# Autodesk Inventor assembly: BG102_trajan20_22
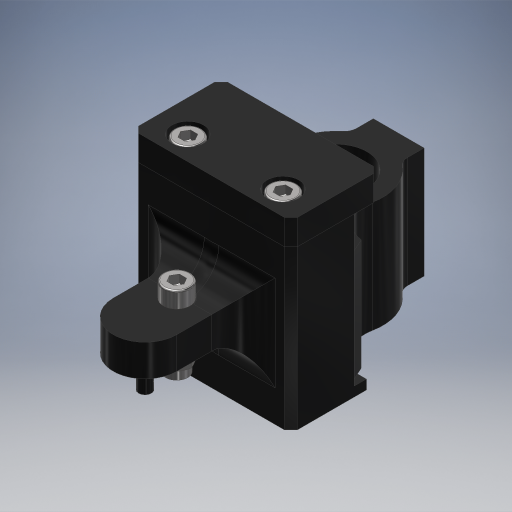
[picture p0: Inventor's stored thumbnail of the model, 512x512]
Saved by Autodesk Inventor 2023 (Build 270158000, 158)
## iProperties
Company: HTBLA Kaindorf
RuleStatus: InUse
Created: 2022-11-06
Part Number: BG102_trajan20_22
Project: Zeichenmaschine_neu
Material: Generisch
Description: Stifthalter
Document SubType Name: Assembly
Designer: trajan20
AfterDocNew0: iProperties-Editor_aufrufen
Author: jan
Keywords: 2022
## Documents named in this file (11)
- C:\Users\jan\Documents\Zeichenmaschine_neu\BG103_trajan20_22_Zeichenmaschine_neu_Stifthalter.iam
- C:\Users\jan\Documents\Zeichenmaschine_neu\BT501_trajan20_21_Zeichenmaschine_v2_Stifthalter außen.ipt
- C:\Users\jan\Documents\Zeichenmaschine_neu\BT502_trajan20_21_Zeichenmaschine_v2_Stifthalter innen.ipt
- C:\Users\jan\Documents\Zeichenmaschine_neu\BT503_trajan20_21_Zeichenmaschine_v2_Stifthalter_platte.ipt
- C:\Users\jan\Documents\Zeichenmaschine_neu\BT504_trajan20_21_Zeichenmaschine_v2_Stifthalter_feder.ipt
- C:\Users\jan\Documents\Zeichenmaschine_neu\Normteile\de-DE\DIN 916\DIN 916 - M5  x  12.ipt
- C:\Users\jan\Documents\Zeichenmaschine_neu\Normteile\de-DE\ISO 4762(2)\ISO 4762 - M5 x 12ISO.ipt
- C:\Users\jan\Documents\Zeichenmaschine_neu\Normteile\de-DE\ISO 4762(2)\ISO 4762 - M5 x 20ISO.ipt
- C:\Users\jan\Documents\Zeichenmaschine_neu\Normteile\de-DE\ISO 10511\ISO 10511 - M5.ipt
- C:\Users\jan\Documents\Zeichenmaschine_neu\Compress Spring11.ipt
- C:\Users\jan\Documents\Zeichenmaschine_neu\Compress Spring12.ipt
## Components (13 placed, 9 different names)
1. BT501_trajan20_21_Zeichenmaschine_v2_Stifthalter außen:1 — Fluchtend:1, Passend:2, Fluchtend:2, Fluchtend:3, Passend:10, Passend:12, Passend:14, Passend:15, Passend:16, Passend:21, Passend:22
2. BT502_trajan20_21_Zeichenmaschine_v2_Stifthalter innen:1 — Fluchtend:1, Passend:4, Passend:5, Passend:6, Passend:7, Passend:8, Passend:9, Fluchtend:4, Fluchtend:5, Passend:19, Fluchtend:7, Passend:20, Fluchtend:8, Passend:21, Passend:22
3. BT503_trajan20_21_Zeichenmaschine_v2_Stifthalter_platte:1 — Passend:2, Fluchtend:2, Fluchtend:3, Passend:11, Passend:13
4. BT504_trajan20_21_Zeichenmaschine_v2_Stifthalter_feder:1 — Passend:6, Passend:7
5. BT504_trajan20_21_Zeichenmaschine_v2_Stifthalter_feder:2 — Passend:4, Passend:5
6. Compress Spring1:1 — Passend:20, Fluchtend:8
7. Compress Spring1:1 — Passend:19, Fluchtend:7
8. DIN 916 M5  x  12:1 — Passend:8, Fluchtend:5
9. DIN 916 M5  x  12:2 — Passend:9, Fluchtend:4
10. ISO 4762 M5 x 12:1 — Passend:10, Passend:11
11. ISO 4762 M5 x 12:2 — Passend:12, Passend:13
12. ISO 4762 M5 x 20:1 — Passend:14, Passend:15, Passend:17
13. DIN EN ISO 10511 M5:1 — Passend:16, Passend:17
## Relationships (26: Mate 19, Flush 7)
- Fluchtend:1 [Flush] (10 mm): BT501_trajan20_21_Zeichenmaschine_v2_Stifthalter außen:1 ↔ BT502_trajan20_21_Zeichenmaschine_v2_Stifthalter innen:1
- Passend:2 [Mate]: BT501_trajan20_21_Zeichenmaschine_v2_Stifthalter außen:1 ↔ BT503_trajan20_21_Zeichenmaschine_v2_Stifthalter_platte:1
- Fluchtend:2 [Flush]: BT501_trajan20_21_Zeichenmaschine_v2_Stifthalter außen:1 ↔ BT503_trajan20_21_Zeichenmaschine_v2_Stifthalter_platte:1
- Fluchtend:3 [Flush]: BT501_trajan20_21_Zeichenmaschine_v2_Stifthalter außen:1 ↔ BT503_trajan20_21_Zeichenmaschine_v2_Stifthalter_platte:1
- Passend:4 [Mate]: BT502_trajan20_21_Zeichenmaschine_v2_Stifthalter innen:1 ↔ BT504_trajan20_21_Zeichenmaschine_v2_Stifthalter_feder:2
- Passend:5 [Mate]: BT502_trajan20_21_Zeichenmaschine_v2_Stifthalter innen:1 ↔ BT504_trajan20_21_Zeichenmaschine_v2_Stifthalter_feder:2
- Passend:6 [Mate]: BT502_trajan20_21_Zeichenmaschine_v2_Stifthalter innen:1 ↔ BT504_trajan20_21_Zeichenmaschine_v2_Stifthalter_feder:1
- Passend:7 [Mate]: BT502_trajan20_21_Zeichenmaschine_v2_Stifthalter innen:1 ↔ BT504_trajan20_21_Zeichenmaschine_v2_Stifthalter_feder:1
- Passend:8 [Mate]: BT502_trajan20_21_Zeichenmaschine_v2_Stifthalter innen:1 ↔ DIN 916 M5  x  12:1
- Passend:9 [Mate]: BT502_trajan20_21_Zeichenmaschine_v2_Stifthalter innen:1 ↔ DIN 916 M5  x  12:2
- Fluchtend:4 [Flush] (3 mm): BT502_trajan20_21_Zeichenmaschine_v2_Stifthalter innen:1 ↔ DIN 916 M5  x  12:2
- Fluchtend:5 [Flush] (3 mm): BT502_trajan20_21_Zeichenmaschine_v2_Stifthalter innen:1 ↔ DIN 916 M5  x  12:1
- Passend:10 [Mate]: BT501_trajan20_21_Zeichenmaschine_v2_Stifthalter außen:1 ↔ ISO 4762 M5 x 12:1
- Passend:11 [Mate]: BT503_trajan20_21_Zeichenmaschine_v2_Stifthalter_platte:1 ↔ ISO 4762 M5 x 12:1
- Passend:12 [Mate]: BT501_trajan20_21_Zeichenmaschine_v2_Stifthalter außen:1 ↔ ISO 4762 M5 x 12:2
- Passend:13 [Mate]: BT503_trajan20_21_Zeichenmaschine_v2_Stifthalter_platte:1 ↔ ISO 4762 M5 x 12:2
- Passend:14 [Mate]: BT501_trajan20_21_Zeichenmaschine_v2_Stifthalter außen:1 ↔ ISO 4762 M5 x 20:1
- Passend:15 [Mate]: BT501_trajan20_21_Zeichenmaschine_v2_Stifthalter außen:1 ↔ ISO 4762 M5 x 20:1
- Passend:16 [Mate] (5 mm): BT501_trajan20_21_Zeichenmaschine_v2_Stifthalter außen:1 ↔ DIN EN ISO 10511 M5:1
- Passend:17 [Mate]: ISO 4762 M5 x 20:1 ↔ DIN EN ISO 10511 M5:1
- Passend:19 [Mate]: BT502_trajan20_21_Zeichenmaschine_v2_Stifthalter innen:1 ↔ Compress Spring1:1
- Fluchtend:7 [Flush]: BT502_trajan20_21_Zeichenmaschine_v2_Stifthalter innen:1 ↔ Compress Spring1:1
- Passend:20 [Mate]: BT502_trajan20_21_Zeichenmaschine_v2_Stifthalter innen:1 ↔ Compress Spring1:1
- Fluchtend:8 [Flush]: BT502_trajan20_21_Zeichenmaschine_v2_Stifthalter innen:1 ↔ Compress Spring1:1
- Passend:21 [Mate]: BT501_trajan20_21_Zeichenmaschine_v2_Stifthalter außen:1 ↔ BT502_trajan20_21_Zeichenmaschine_v2_Stifthalter innen:1
- Passend:22 [Mate]: BT501_trajan20_21_Zeichenmaschine_v2_Stifthalter außen:1 ↔ BT502_trajan20_21_Zeichenmaschine_v2_Stifthalter innen:1
